# Autodesk Inventor assembly: test 1
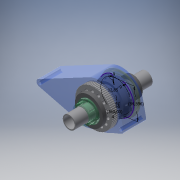
[picture p0: Inventor's stored thumbnail of the model, 180x180]
Saved by Autodesk Inventor 2018.1 (Build 221171000, 171)
## iProperties
Created: 2022-07-20
Part Number: test 1
Document SubType Name: Assembly
Designer: mouta
Author: mouta
## Documents named in this file (3)
- C:\Users\mouta\GoogleDrive\Manu\USINAGE\MoteurVelo\test 1.iam
- C:\Users\mouta\GoogleDrive\Manu\USINAGE\MoteurVelo\Corps\body depart.ipt
- C:\Users\mouta\GoogleDrive\Manu\USINAGE\MoteurVelo\Arbre primaire\Assembly1.iam
## Components (2 placed, 2 different names)
1. body depart:1 — Mate:1, Flush:1
2. Assembly1:1 [sub-assembly] — Mate:1, Flush:1
## Relationships (2: Mate 1, Flush 1)
- Mate:1: body depart:1 ↔ Assembly1:1
- Flush:1 (45 mm): body depart:1 ↔ Assembly1:1
